# Autodesk Inventor assembly: base
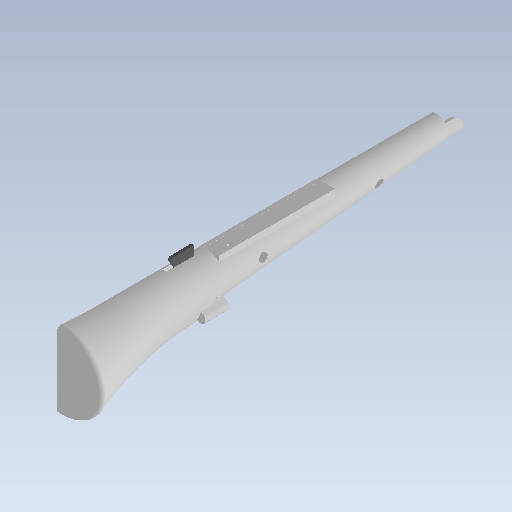
[picture p0: Inventor's stored thumbnail of the model, 512x512]
Saved by Autodesk Inventor 2021 (Build 250183000, 183)
## iProperties
Created: 2023-09-03
Part Number: base
Document SubType Name: Assembly
Designer: Sergio
Mass: 360.631 g
Surface Area: 1399.84 cm^2
Volume: 339.274 cm^3
Density: 1.06295 g/cm^3
Author: Sergio
## Documents named in this file (8)
- D:\Sergio\OneDrive - Escuela Superior Politécnica del Litoral\Documentos\12vo Semestre (último)\Diseño Mecatrónico\Proyecto\Diseño Mecánico\solucion GANADORA\Base\base.iam
- D:\Sergio\OneDrive - Escuela Superior Politécnica del Litoral\Documentos\12vo Semestre (último)\Diseño Mecatrónico\Proyecto\Diseño Mecánico\solucion GANADORA\trigger_mechanism\Mecanismo de Gatillo.iam
- D:\Sergio\Documents\Inventor\Content Center Files\R2021\es-ES\ANSI B 18.6.7 M IFI 513(2)\ANSI B 18.6.7 M _ IFI 513 - M4x0.7 x 12(1).ipt
- D:\Sergio\Documents\Inventor\Content Center Files\R2021\es-ES\AS 1427(04)\AS 1427 - M4 x 20(5) I.ipt
- D:\Sergio\Documents\Inventor\Content Center Files\R2021\es-ES\DIN 7985 (H)\DIN 7985 (H) - M4x10-H.ipt
- D:\Sergio\OneDrive - Escuela Superior Politécnica del Litoral\Documentos\12vo Semestre (último)\Diseño Mecatrónico\Proyecto\Diseño Mecánico\solucion GANADORA\Base\Base superior derecha.ipt
- D:\Sergio\OneDrive - Escuela Superior Politécnica del Litoral\Documentos\12vo Semestre (último)\Diseño Mecatrónico\Proyecto\Diseño Mecánico\solucion GANADORA\Base\Base superior izquierda.ipt
- D:\Sergio\OneDrive - Escuela Superior Politécnica del Litoral\Documentos\12vo Semestre (último)\Diseño Mecatrónico\Proyecto\Diseño Mecánico\solucion GANADORA\Base\Base sección inferior.ipt
## Components (9 placed, 7 different names)
1. Base sección inferior:1 — Coincidencia:1, Coincidencia:2, Coincidencia:3, Nivelación:1, Coincidencia:6, Coincidencia:7, Coincidencia:10, Insertar:1, Coincidencia:15, Nivelación:2, Nivelación:3
2. Base superior izquierda:1 — Coincidencia:13, Coincidencia:14, Coincidencia:15, Coincidencia:16
3. Base superior derecha:1 — Coincidencia:6, Coincidencia:7, Coincidencia:8, Coincidencia:9, Coincidencia:11, Coincidencia:12, Coincidencia:13, Coincidencia:14, Insertar:2, Insertar:3
4. Mecanismo de Gatillo:1 [sub-assembly] — Coincidencia:1, Coincidencia:4, Coincidencia:9, Coincidencia:11, Coincidencia:12
5. Tornillo para maquinaria de cabeza hex. bridada - Métrico M4x0.7 x 12:1 — Coincidencia:2, Coincidencia:3, Coincidencia:4
6. AS 1427 H - Métrico M4 x 20:1 — Coincidencia:8, Coincidencia:10, Insertar:1
7. AS 1427 H - Métrico M4 x 20:2 — Coincidencia:16
8. DIN 7985 (H) M4x10-H:2 — Insertar:2
9. DIN 7985 (H) M4x10-H:1 — Insertar:3
## Relationships (21: Mate 15, Flush 3, Insert 3)
- Coincidencia:1 [Mate]: Base sección inferior:1 ↔ Mecanismo de Gatillo:1
- Coincidencia:2 [Mate]: Base sección inferior:1 ↔ Tornillo para maquinaria de cabeza hex. bridada - Métrico M4x0.7 x 12:1
- Coincidencia:3 [Mate]: Base sección inferior:1 ↔ Tornillo para maquinaria de cabeza hex. bridada - Métrico M4x0.7 x 12:1
- Coincidencia:4 [Mate]: Mecanismo de Gatillo:1 ↔ Tornillo para maquinaria de cabeza hex. bridada - Métrico M4x0.7 x 12:1
- Nivelación:1 [Flush]: Base sección inferior:1
- Coincidencia:6 [Mate]: Base sección inferior:1 ↔ Base superior derecha:1
- Coincidencia:7 [Mate]: Base sección inferior:1 ↔ Base superior derecha:1
- Coincidencia:8 [Mate]: Base superior derecha:1 ↔ AS 1427 H - Métrico M4 x 20:1
- Coincidencia:9 [Mate]: Base superior derecha:1 ↔ Mecanismo de Gatillo:1
- Coincidencia:10 [Mate]: Base sección inferior:1 ↔ AS 1427 H - Métrico M4 x 20:1
- Insertar:1: Base sección inferior:1 ↔ AS 1427 H - Métrico M4 x 20:1
- Coincidencia:11 [Mate]: Base superior derecha:1 ↔ Mecanismo de Gatillo:1
- Coincidencia:12 [Mate]: Base superior derecha:1 ↔ Mecanismo de Gatillo:1
- Coincidencia:13 [Mate]: Base superior izquierda:1 ↔ Base superior derecha:1
- Coincidencia:14 [Mate]: Base superior izquierda:1 ↔ Base superior derecha:1
- Coincidencia:15 [Mate]: Base sección inferior:1 ↔ Base superior izquierda:1
- Coincidencia:16 [Mate]: Base superior izquierda:1 ↔ AS 1427 H - Métrico M4 x 20:2
- Insertar:2: Base superior derecha:1 ↔ DIN 7985 (H) M4x10-H:2
- Insertar:3: Base superior derecha:1 ↔ DIN 7985 (H) M4x10-H:1
- Nivelación:2 [Flush]: Base sección inferior:1
- Nivelación:3 [Flush]: Base sección inferior:1
